# Autodesk Inventor assembly: LCD-1234-SA
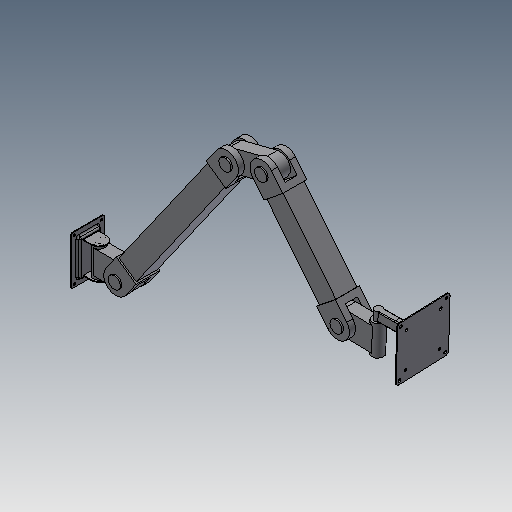
[picture p0: Inventor's stored thumbnail of the model, 512x512]
Saved by Autodesk Inventor 2018.3 (Build 223284000, 284)
## iProperties
Created: 2004-11-28
Part Number: LCD-1234-SA
Document SubType Name: Assembly
Designer: Autodesk, Inc.
Manufacturer: Standard
Standards Organization: Custom
Description: SWING ARM, LCD FLAT PANEL
Mass: 1844.58 g
Surface Area: 2731.03 cm^2
Volume: 1844.58 cm^3
Density: 1 g/cm^3
CAGE: 1LJX3
Dept. ID: Product Design
Description #2: ---
Finish #1: ---
Finish #2: ---
Material ID: ---
Project Number: ---
Author: Autodesk, Inc.
## Documents named in this file (7)
- C:\AVAInvAPI\Workspace\Test Station\Components\SwingArm.iam
- C:\AVAInvAPI\Workspace\Test Station\Components\BasePivot.ipt
- C:\AVAInvAPI\Workspace\Test Station\Components\LongArm.ipt
- C:\AVAInvAPI\Workspace\Test Station\Components\Joint.ipt
- C:\AVAInvAPI\Workspace\Test Station\Components\ShortArm.ipt
- C:\AVAInvAPI\Workspace\Test Station\Components\MonitorMount.ipt
- C:\AVAInvAPI\Workspace\Test Station\Components\WallMount.ipt
## Components (7 placed, 6 different names)
1. WallMount:1 — Insert:6, Angle:1
2. BasePivot:1 — Insert:1, Insert:6, Angle:1
3. LongArm:1 — Insert:1, Insert:2
4. Joint:1 — Insert:2, Insert:3
5. ShortArm:1 — Insert:3, Insert:4
6. BasePivot:2 — Insert:4, Insert:5
7. MonitorMount:1 — Insert:5
## Relationships (7: Insert 6, Angle 1)
- Insert:1: BasePivot:1 ↔ LongArm:1
- Insert:2: LongArm:1 ↔ Joint:1
- Insert:3: Joint:1 ↔ ShortArm:1
- Insert:4: ShortArm:1 ↔ BasePivot:2
- Insert:5: BasePivot:2 ↔ MonitorMount:1
- Insert:6: WallMount:1 ↔ BasePivot:1
- Angle:1 (0 deg): WallMount:1 ↔ BasePivot:1
